# Autodesk Inventor assembly: Ensamblaje
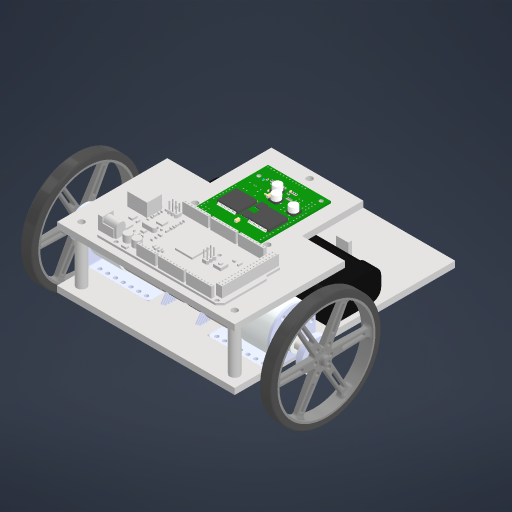
[picture p0: Inventor's stored thumbnail of the model, 512x512]
Saved by Autodesk Inventor 2023 (Build 270158000, 158)
## iProperties
Created: 2022-08-21
Part Number: Ensamblaje
Document SubType Name: Assembly
Designer: marat
Author: marat
## Documents named in this file (15)
- C:\Users\marat\Documents\IRB2001\Ensamblaje.iam
- C:\Users\marat\Documents\IRB2001\chasis.ipt
- C:\Users\marat\Documents\IRB2001\Piezas 3D Robot\Bateria.ipt
- C:\Users\marat\Documents\IRB2001\Piezas 3D Robot\pololu-stamped-aluminum-l-bracket-for-37d-mm-metal-gearmotors.ipt
- C:\Users\marat\Documents\IRB2001\Piezas 3D Robot\37d-gearmotor-50-70-encoder.ipt
- C:\Users\marat\Documents\IRB2001\Piezas 3D Robot\pololu-wheel-90x10mm-black.ipt
- C:\Users\marat\Documents\IRB2001\Piezas 3D Robot\pololu-universal-aluminum-mounting-hub-for-6mm-shaft-4-40-holes.ipt
- C:\Users\marat\Documents\IRB2001\Piezas 3D Robot\pololu-stamped-aluminum-l-bracket-for-37d-mm-metal-gearmotors_MIR.ipt
- C:\Users\marat\Documents\IRB2001\Piezas 3D Robot\37d-gearmotor-50-70-encoder_MIR1.ipt
- C:\Users\marat\Documents\IRB2001\Piezas 3D Robot\pololu-wheel-90x10mm-black_MIR.ipt
- C:\Users\marat\Documents\IRB2001\Piezas 3D Robot\pololu-universal-aluminum-mounting-hub-for-6mm-shaft-4-40-holes_MIR.ipt
- C:\Users\marat\Documents\IRB2001\pilar.ipt
- C:\Users\marat\Documents\IRB2001\chasis_arriba.ipt
- C:\Users\marat\Documents\IRB2001\Piezas 3D Robot\ArduinoMega_STEP_AP203.ipt
- C:\Users\marat\Documents\IRB2001\Piezas 3D Robot\pololu-dual-vnh5019-motor-driver-shield.ipt
## Components (18 placed, 14 different names)
1. chasis:1 — Mate:24, Mate:25, Mate:26, Mate:27, Mate:29, Mate:30, Mate:32, Mate:33, Mate:34, Mate:36, Mate:40
2. Bateria:1 — Mate:29, Mate:30
3. pololu-stamped-aluminum-l-bracket-for-37d-mm-metal-gearmotors:1 — Mate:1, Mate:6, Mate:27
4. 37d-gearmotor-50-70-encoder:2 — Mate:1, Mate:3, Flush:1, Mate:6, Flush:4, Flush:5
5. pololu-wheel-90x10mm-black:1 — Mate:5, Mate:7, Mate:8
6. pololu-universal-aluminum-mounting-hub-for-6mm-shaft-4-40-holes:2 — Mate:3, Flush:1, Mate:5, Mate:7, Mate:8
7. pololu-stamped-aluminum-l-bracket-for-37d-mm-metal-gearmotors_MIR:1 — Mate:15, Mate:16, Mate:24, Mate:25, Mate:26
8. 37d-gearmotor-50-70-encoder_MIR1:1 — Mate:15, Mate:16, Flush:3, Mate:20, Flush:4, Flush:5
9. pololu-wheel-90x10mm-black_MIR:1 — Mate:17, Mate:18, Mate:19
10. pololu-universal-aluminum-mounting-hub-for-6mm-shaft-4-40-holes_MIR:1 — Mate:17, Mate:18, Mate:19, Flush:3, Mate:20
11. pilar:1 — Mate:36, Mate:37
12. pilar:2 — Mate:32
13. pilar:3 — Mate:33
14. pilar:4 — Mate:34
15. pilar:5 — Mate:40
16. chasis_arriba:1 — Mate:37, Mate:38, Mate:39
17. ArduinoMega_STEP_AP203:1 — Mate:38
18. pololu-dual-vnh5019-motor-driver-shield:1 — Mate:39
## Relationships (30: Mate 26, Flush 4)
- Mate:1: pololu-stamped-aluminum-l-bracket-for-37d-mm-metal-gearmotors:1 ↔ 37d-gearmotor-50-70-encoder:2
- Mate:3: 37d-gearmotor-50-70-encoder:2 ↔ pololu-universal-aluminum-mounting-hub-for-6mm-shaft-4-40-holes:2
- Flush:1: 37d-gearmotor-50-70-encoder:2 ↔ pololu-universal-aluminum-mounting-hub-for-6mm-shaft-4-40-holes:2
- Mate:5: pololu-wheel-90x10mm-black:1 ↔ pololu-universal-aluminum-mounting-hub-for-6mm-shaft-4-40-holes:2
- Mate:6: pololu-stamped-aluminum-l-bracket-for-37d-mm-metal-gearmotors:1 ↔ 37d-gearmotor-50-70-encoder:2
- Mate:7: pololu-wheel-90x10mm-black:1 ↔ pololu-universal-aluminum-mounting-hub-for-6mm-shaft-4-40-holes:2
- Mate:8: pololu-wheel-90x10mm-black:1 ↔ pololu-universal-aluminum-mounting-hub-for-6mm-shaft-4-40-holes:2
- Mate:15: pololu-stamped-aluminum-l-bracket-for-37d-mm-metal-gearmotors_MIR:1 ↔ 37d-gearmotor-50-70-encoder_MIR1:1
- Mate:16: pololu-stamped-aluminum-l-bracket-for-37d-mm-metal-gearmotors_MIR:1 ↔ 37d-gearmotor-50-70-encoder_MIR1:1
- Mate:17: pololu-wheel-90x10mm-black_MIR:1 ↔ pololu-universal-aluminum-mounting-hub-for-6mm-shaft-4-40-holes_MIR:1
- Mate:18: pololu-wheel-90x10mm-black_MIR:1 ↔ pololu-universal-aluminum-mounting-hub-for-6mm-shaft-4-40-holes_MIR:1
- Mate:19: pololu-wheel-90x10mm-black_MIR:1 ↔ pololu-universal-aluminum-mounting-hub-for-6mm-shaft-4-40-holes_MIR:1
- Flush:3: 37d-gearmotor-50-70-encoder_MIR1:1 ↔ pololu-universal-aluminum-mounting-hub-for-6mm-shaft-4-40-holes_MIR:1
- Mate:20: 37d-gearmotor-50-70-encoder_MIR1:1 ↔ pololu-universal-aluminum-mounting-hub-for-6mm-shaft-4-40-holes_MIR:1
- Flush:4: 37d-gearmotor-50-70-encoder:2 ↔ 37d-gearmotor-50-70-encoder_MIR1:1
- Flush:5: 37d-gearmotor-50-70-encoder:2 ↔ 37d-gearmotor-50-70-encoder_MIR1:1
- Mate:24: chasis:1 ↔ pololu-stamped-aluminum-l-bracket-for-37d-mm-metal-gearmotors_MIR:1
- Mate:25: chasis:1 ↔ pololu-stamped-aluminum-l-bracket-for-37d-mm-metal-gearmotors_MIR:1
- Mate:26: chasis:1 ↔ pololu-stamped-aluminum-l-bracket-for-37d-mm-metal-gearmotors_MIR:1
- Mate:27: chasis:1 ↔ pololu-stamped-aluminum-l-bracket-for-37d-mm-metal-gearmotors:1
- Mate:29: chasis:1 ↔ Bateria:1
- Mate:30: chasis:1 ↔ Bateria:1
- Mate:32: chasis:1 ↔ pilar:2
- Mate:33: chasis:1 ↔ pilar:3
- Mate:34: chasis:1 ↔ pilar:4
- Mate:36: chasis:1 ↔ pilar:1
- Mate:37: pilar:1 ↔ chasis_arriba:1
- Mate:38: chasis_arriba:1 ↔ ArduinoMega_STEP_AP203:1
- Mate:39: chasis_arriba:1 ↔ pololu-dual-vnh5019-motor-driver-shield:1
- Mate:40: chasis:1 ↔ pilar:5
